# Autodesk Inventor assembly: R-wing
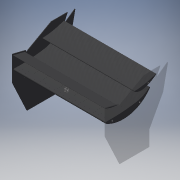
[picture p0: Inventor's stored thumbnail of the model, 180x180]
Saved by Autodesk Inventor 2018.2 (Build 222227000, 227)
## iProperties
Created: 2017-12-11
Part Number: R-wing
Material: 一般
Document SubType Name: Assembly
Designer: kuwano
Mass: 31755.7 g
Surface Area: 41187.6 cm^2
Volume: 30692.1 cm^3
Density: 1.03465 g/cm^3
Author: kuwano
## Documents named in this file (5)
- Z:\各班フォルダ\2018\ボディ\カウル\AeroCAD2018\CAD\Inventor\製作用CAD\R-wing\R-wing.iam
- Z:\各班フォルダ\2018\ボディ\カウル\AeroCAD2018\CAD\Inventor\製作用CAD\R-wing\parts\main_flap\main_flap.iam
- Z:\各班フォルダ\2018\ボディ\カウル\AeroCAD2018\CAD\Inventor\製作用CAD\R-wing\parts\end_plate.ipt
- Z:\各班フォルダ\2018\ボディ\カウル\AeroCAD2018\CAD\Inventor\製作用CAD\R-wing\parts\sub_flap\sub_flap.iam
- Z:\各班フォルダ\2018\ボディ\カウル\AeroCAD2018\CAD\Inventor\製作用CAD\R-wing\parts\foward_flap.ipt
## Components (5 placed, 4 different names)
1. main_flap:1 [sub-assembly] — メイト:1, メイト:2, メイト:13, メイト:15
2. sub_flap:1 [sub-assembly] — メイト:14, メイト:16
3. end_plate:1 — メイト:1, フラッシュ:1, フラッシュ:2, メイト:14, メイト:15, メイト:16, メイト:17, 角度:1, フラッシュ:3
4. end_plate:2 — メイト:2, フラッシュ:1, フラッシュ:2, メイト:13
5. foward_flap:1 — メイト:17, 角度:1, フラッシュ:3
## Relationships (11: Mate 7, Flush 3, Angle 1)
- メイト:1 [Mate]: main_flap:1 ↔ end_plate:1
- メイト:2 [Mate]: main_flap:1 ↔ end_plate:2
- フラッシュ:1 [Flush]: end_plate:1 ↔ end_plate:2
- フラッシュ:2 [Flush]: end_plate:1 ↔ end_plate:2
- メイト:13 [Mate]: main_flap:1 ↔ end_plate:2
- メイト:14 [Mate]: sub_flap:1 ↔ end_plate:1
- メイト:15 [Mate]: main_flap:1 ↔ end_plate:1
- メイト:16 [Mate]: sub_flap:1 ↔ end_plate:1
- メイト:17 [Mate]: end_plate:1 ↔ foward_flap:1
- 角度:1 [Angle] (0 deg): end_plate:1 ↔ foward_flap:1
- フラッシュ:3 [Flush] (10 mm): end_plate:1 ↔ foward_flap:1
